# Autodesk Inventor assembly: Assembly
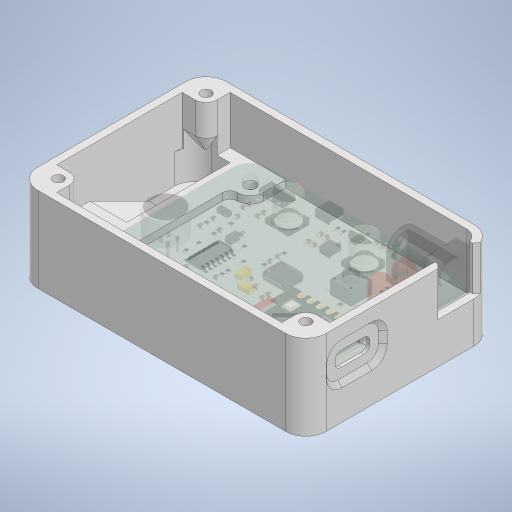
[picture p0: Inventor's stored thumbnail of the model, 512x512]
Saved by Autodesk Inventor 2023 (Build 270158000, 158)
## iProperties
Created: 2024-10-10
Part Number: Assembly
Document SubType Name: Assembly
Designer: noname
Author: noname
## Documents named in this file (6)
- C:\Users\noname\Documents\GitHub\Seismometer-esp32\Case\Assembly.iam
- C:\Users\noname\Documents\GitHub\Seismometer-esp32\Case\seismometer-esp32.ipt
- C:\Users\noname\Documents\GitHub\Seismometer-esp32\Case\Main body.ipt
- C:\Users\noname\Documents\GitHub\Seismometer-esp32\Case\35mm-sensor.ipt
- C:\Users\noname\Documents\GitHub\Seismometer-esp32\Case\Part1.ipt
- C:\Users\noname\Documents\GitHub\Seismometer-esp32\Case\Part2.ipt
## Components (5 placed, 5 different names)
1. seismometer-esp32:1 — Rotational:1, Angle:1
2. Main body:1 — Rotational:1, Angle:1, Cylindrical:1, Mate:1, Flush:1
3. 35mm-sensor:1 — Cylindrical:1, Mate:1
4. Part1:1 — Flush:1, Flush:2
5. Part2:1 — Flush:2
## Relationships (6: Flush 2, RevoluteJoint 1, Angle 1, CylindricalJoint 1, Mate 1)
- Rotational:1 [RevoluteJoint]: seismometer-esp32:1 ↔ Main body:1
- Angle:1 (180 deg): seismometer-esp32:1 ↔ Main body:1
- Cylindrical:1: Main body:1 ↔ 35mm-sensor:1
- Mate:1 (0.5 mm): Main body:1 ↔ 35mm-sensor:1
- Flush:1: Main body:1 ↔ Part1:1
- Flush:2: Part1:1 ↔ Part2:1
